# Autodesk Inventor assembly: small caster
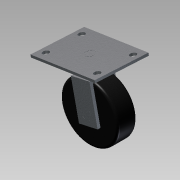
[picture p0: Inventor's stored thumbnail of the model, 180x180]
Saved by Autodesk Inventor 2012 (Build 160160000, 160)
## iProperties
Created: 2012-09-15
Part Number: small caster
Document SubType Name: Assembly
Designer: Admin
Author: Admin
## Documents named in this file (4)
- C:\Users\Admin\Documents\Inventor\Robotics 2013\Cart\small caster\small caster.iam
- C:\Users\Admin\Documents\Inventor\Robotics 2013\Cart\small caster\rubber wheel.ipt
- C:\Users\Admin\Documents\Inventor\Robotics 2013\Cart\small caster\small wheel support.ipt
- C:\Users\Admin\Documents\Inventor\Robotics 2013\Cart\small caster\mount plate.ipt
## Components (3 placed, 3 different names)
1. rubber wheel:1 — Mate:1, Flush:1
2. small wheel support:1 — Mate:1, Flush:1, Flush:2, Mate:2
3. mount plate:1 — Flush:2, Mate:2
## Relationships (4: Mate 2, Flush 2)
- Mate:1: rubber wheel:1 ↔ small wheel support:1
- Flush:1: rubber wheel:1 ↔ small wheel support:1
- Flush:2: small wheel support:1 ↔ mount plate:1
- Mate:2: small wheel support:1 ↔ mount plate:1
